# Autodesk Inventor assembly: Pre-roller
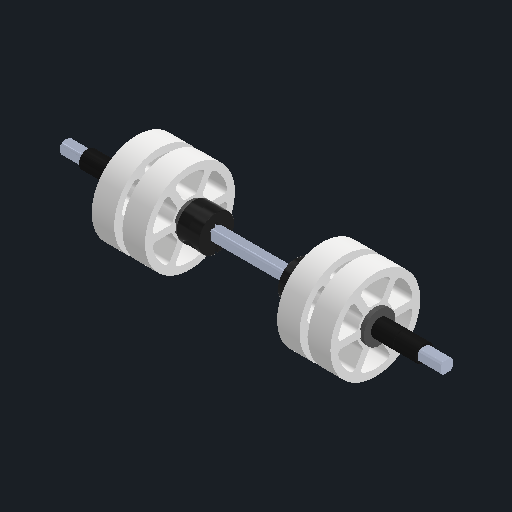
[picture p0: Inventor's stored thumbnail of the model, 512x512]
Saved by Autodesk Inventor 2025 (Build 290162000, 162)
## iProperties
Created: 2024-10-21
Part Number: Pre-roller
Document SubType Name: Assembly
Designer: averey
Author: averey
## Documents named in this file (7)
- D:\VEX\High Stakes\CAD\V2\Intake\Floating Stage\Pre-roller.iam
- D:\VEX\High Stakes\CAD\ROBOPROS-CAD-Inventor\Motion\Shaft HS\Shaft HS\Shaft HS 8.5 in.ipt
- C:\Users\avere\VEX\High Stakes\CAD\ROBOPROS-CAD-Inventor\Motion\Shaft HS\Shaft HS.ipt
- D:\VEX\High Stakes\CAD\ROBOPROS-CAD-Inventor\Quick Assemblies\2.000 30A .500 With Adapters.iam
- D:\VEX\High Stakes\CAD\ROBOPROS-CAD-Inventor\Motion\Shaft HS\HS Spacer\HSpacer .5000.ipt
- C:\Users\avere\VEX\High Stakes\CAD\ROBOPROS-CAD-Inventor\Motion\Shaft HS\HS Spacer.ipt
- D:\VEX\High Stakes\CAD\ROBOPROS-CAD-Inventor\Motion\Shaft HS\HS Shaft Collar.ipt
## Components (11 placed, 4 different names)
1. Shaft HS 8.5 in:1 — Flush:1, Mate:1, Mate:2, Insert:3, Flush:2
2. 2.000 30A .500 With Adapters:1 [sub-assembly] — Insert:1, Mate:3, Insert:8
3. 2.000 30A .500 With Adapters:2 [sub-assembly] — Insert:1, Insert:3, Insert:5
4. 2.000 30A .500 With Adapters:3 [sub-assembly] — Insert:9
5. 2.000 30A .500 With Adapters:4 [sub-assembly] — Mate:3, Flush:2, Insert:7
6. HSpacer .5000:1 — Insert:4, Insert:5
7. HSpacer .5000:2 — Insert:4
8. HSpacer .5000:3
9. HSpacer .5000:4 — Insert:7
10. HS Shaft Collar:1 — Insert:9
11. HS Shaft Collar:2 — Insert:8
## Relationships (14: Insert 9, Mate 3, Flush 2)
- Flush:1 (-107.95 mm): Shaft HS 8.5 in:1
- Mate:1: Shaft HS 8.5 in:1
- Mate:2: Shaft HS 8.5 in:1
- Insert:1: 2.000 30A .500 With Adapters:1 ↔ 2.000 30A .500 With Adapters:2
- [Insert]: 2.000 30A .500 With Adapters:3 ↔ 2.000 30A .500 With Adapters:4
- Insert:3 (38.1 mm): Shaft HS 8.5 in:1 ↔ 2.000 30A .500 With Adapters:2
- Mate:3: 2.000 30A .500 With Adapters:1 ↔ 2.000 30A .500 With Adapters:4
- Flush:2 (38.1 mm): Shaft HS 8.5 in:1 ↔ 2.000 30A .500 With Adapters:4
- Insert:4: HSpacer .5000:1 ↔ HSpacer .5000:2
- Insert:5: 2.000 30A .500 With Adapters:2 ↔ HSpacer .5000:1
- [Insert]: HSpacer .5000:3 ↔ HSpacer .5000:4
- Insert:7: 2.000 30A .500 With Adapters:4 ↔ HSpacer .5000:4
- Insert:8: 2.000 30A .500 With Adapters:1 ↔ HS Shaft Collar:2
- Insert:9: 2.000 30A .500 With Adapters:3 ↔ HS Shaft Collar:1
## Named parameters: d4_d3 = 0 mm, d10_d8 = 0 mm
